# Autodesk Inventor assembly: ASM
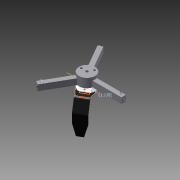
[picture p0: Inventor's stored thumbnail of the model, 180x180]
Saved by Autodesk Inventor 2011 SP2 (Build 150309200, 309)
## iProperties
Created: 2013-02-08
Part Number: ASM
Document SubType Name: Assembly
Designer: sungwook
Author: sungwook
## Documents named in this file (7)
- C:\Users\sungwook\Documents\Inventor\Micron22_top_adj_02082013\02082012_Fiducail_Markers\ASM.iam
- C:\Users\sungwook\Documents\Inventor\Micron22_top_adj_02082013\Parts\Tool\Tool Mount_Rev.ipt
- C:\Users\sungwook\Documents\Inventor\Micron22_top_adj_02082013\02082012_Fiducail_Markers\Fiducial_Post.ipt
- C:\Users\sungwook\Documents\Inventor\Micron22_top_adj_02082013\Parts\Main\Platform_Top_14mm_Rev.ipt
- C:\Users\sungwook\Documents\Inventor\Micron22_top_adj_02082013\02082012_Fiducail_Markers\Short_Needle.ipt
- C:\Users\sungwook\Documents\Inventor\Content Center Files\R2011\en-US\ANSI B18.3(18)\ANSI B18.3 - 0-80 UNF - 0.13(28).ipt
- C:\Users\sungwook\Documents\Inventor\Micron22_top_adj_02082013\Parts\ASAP\ASAP_Top_Fixture_New.ipt
## Components (10 placed, 6 different names)
1. Platform_Top_14mm_Rev:1 — Mate:9, Mate:10, Mate:11, Mate:19, Mate:20, Mate:21, Mate:22
2. Tool Mount_Rev:1 — Mate:9, Mate:10, Mate:11, Mate:15, Mate:16, Mate:17, Mate:18, Mate:22, Mate:23
3. Fiducial_Post:1 — Mate:12, Mate:13, Mate:14, Flush:1, Mate:15, Mate:16, Mate:17, Mate:18
4. ASAP_Top_Fixture_New:1 — Mate:19, Mate:20, Mate:21, Mate:23
5. Short_Needle:1 — Mate:12, Mate:13
6. Type A - Hexagon Socket Set Screw - Cup Point - Inch 0-80 UNF x 0.13:1 — Mate:14, Flush:1
7. Short_Needle:2
8. Type A - Hexagon Socket Set Screw - Cup Point - Inch 0-80 UNF x 0.13:2
9. Short_Needle:3
10. Type A - Hexagon Socket Set Screw - Cup Point - Inch 0-80 UNF x 0.13:3
## Component patterns: (3 elements, first: Short_Needle:1 + Type A - Hexagon Socket Set Screw - Cup Point - Inch 0-80 UNF x 0.13:1)
## Relationships (16: Mate 15, Flush 1)
- Mate:9: Platform_Top_14mm_Rev:1 ↔ Tool Mount_Rev:1
- Mate:10: Platform_Top_14mm_Rev:1 ↔ Tool Mount_Rev:1
- Mate:11: Platform_Top_14mm_Rev:1 ↔ Tool Mount_Rev:1
- Mate:12: Fiducial_Post:1 ↔ Short_Needle:1
- Mate:13: Fiducial_Post:1 ↔ Short_Needle:1
- Flush:1 (-0.5 mm): Fiducial_Post:1 ↔ Type A - Hexagon Socket Set Screw - Cup Point - Inch 0-80 UNF x 0.13:1
- Mate:15: Tool Mount_Rev:1 ↔ Fiducial_Post:1
- Mate:16: Tool Mount_Rev:1 ↔ Fiducial_Post:1
- Mate:17: Tool Mount_Rev:1 ↔ Fiducial_Post:1
- Mate:18: Tool Mount_Rev:1 ↔ Fiducial_Post:1
- Mate:19: Platform_Top_14mm_Rev:1 ↔ ASAP_Top_Fixture_New:1
- Mate:20: Platform_Top_14mm_Rev:1 ↔ ASAP_Top_Fixture_New:1
- Mate:21: Platform_Top_14mm_Rev:1 ↔ ASAP_Top_Fixture_New:1
- Mate:22: Platform_Top_14mm_Rev:1 ↔ Tool Mount_Rev:1
- Mate:23: Tool Mount_Rev:1 ↔ ASAP_Top_Fixture_New:1
- Mate:14: Fiducial_Post:1 ↔ Type A - Hexagon Socket Set Screw - Cup Point - Inch 0-80 UNF x 0.13:1
